# Autodesk Inventor assembly: Linear-Rail
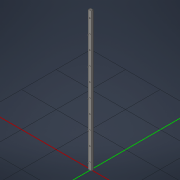
[picture p0: Inventor's stored thumbnail of the model, 180x180]
Saved by Autodesk Inventor 2022.2 (Build 262287010, 287A)
## iProperties
Created: 2022-03-14
Part Number: Linear-Rail
Document SubType Name: Assembly
Designer: sleib
Author: sleib
## Documents named in this file (3)
- C:\Users\sleib\Projekte\Voron-2\CAD\Inventor\Linear-Rail.iam
- C:\Users\sleib\Projekte\Voron-2\CAD\Inventor\MGN9H Linear-Rail (400mm).ipt
- C:\Users\sleib\Projekte\Voron-2\CAD\Inventor\M3x8 SHCS.ipt
## Components (6 placed, 2 different names)
1. MGN9H Linear-Rail (400mm):1 — Passend:1, Passend:2, Passend:3, Passend:4, Passend:5, Passend:6, Passend:7, Passend:8, Passend:9, Passend:10
2. M3x8 SHCS:1 — Passend:1, Passend:6
3. M3x8 SHCS:2 — Passend:2, Passend:7
4. M3x8 SHCS:3 — Passend:3, Passend:8
5. M3x8 SHCS:4 — Passend:4, Passend:9
6. M3x8 SHCS:5 — Passend:5, Passend:10
## Relationships (10: Mate 10)
- Passend:1 [Mate]: MGN9H Linear-Rail (400mm):1 ↔ M3x8 SHCS:1
- Passend:2 [Mate]: MGN9H Linear-Rail (400mm):1 ↔ M3x8 SHCS:2
- Passend:3 [Mate]: MGN9H Linear-Rail (400mm):1 ↔ M3x8 SHCS:3
- Passend:4 [Mate]: MGN9H Linear-Rail (400mm):1 ↔ M3x8 SHCS:4
- Passend:5 [Mate]: MGN9H Linear-Rail (400mm):1 ↔ M3x8 SHCS:5
- Passend:6 [Mate]: MGN9H Linear-Rail (400mm):1 ↔ M3x8 SHCS:1
- Passend:7 [Mate]: MGN9H Linear-Rail (400mm):1 ↔ M3x8 SHCS:2
- Passend:8 [Mate]: MGN9H Linear-Rail (400mm):1 ↔ M3x8 SHCS:3
- Passend:9 [Mate]: MGN9H Linear-Rail (400mm):1 ↔ M3x8 SHCS:4
- Passend:10 [Mate]: MGN9H Linear-Rail (400mm):1 ↔ M3x8 SHCS:5
